# Autodesk Inventor assembly: 部件1
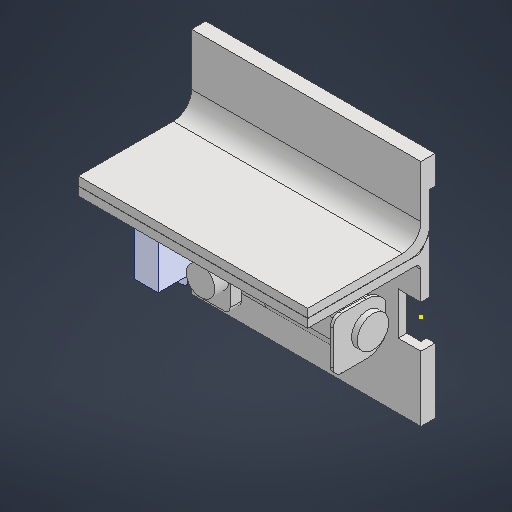
[picture p0: Inventor's stored thumbnail of the model, 512x512]
Saved by Autodesk Inventor 2025 (Build 290162000, 162)
## iProperties
Created: 2025-11-30
Part Number: 部件1
Document SubType Name: Assembly
Designer: XH
Author: XH
## Documents named in this file (6)
- C:\1A_Engineering_files\braille-printer-v2\部件1.iam
- C:\1A_Engineering_files\braille-printer-v2\便签.ipt
- C:\1A_Engineering_files\braille-printer-v2\主体.ipt
- C:\1A_Engineering_files\braille-printer-v2\前舵机位置控制.ipt
- C:\1A_Engineering_files\braille-printer-v2\针头主体.iam
- C:\1A_Engineering_files\braille-printer-v2\电机.ipt
## Components (5 placed, 5 different names)
1. 便签:1 — 配合:1, 配合:2, 配合:3
2. 主体:1 — 配合:1, 配合:2, 表面齐平:1
3. 前舵机位置控制:1 — 配合:3, 表面齐平:1, 配合:4
4. 针头主体:1 [sub-assembly] — 配合:4
5. 电机:1
## Relationships (5: Mate 4, Flush 1)
- 配合:1 [Mate]: 便签:1 ↔ 主体:1
- 配合:2 [Mate]: 便签:1 ↔ 主体:1
- 配合:3 [Mate]: 便签:1 ↔ 前舵机位置控制:1
- 表面齐平:1 [Flush]: 主体:1 ↔ 前舵机位置控制:1
- 配合:4 [Mate]: 前舵机位置控制:1 ↔ 针头主体:1
